# Autodesk Inventor assembly: 200-60-DIFFERENTIAL-BAR-02
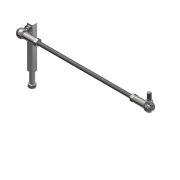
[picture p0: Inventor's stored thumbnail of the model, 180x180]
Saved by Autodesk Inventor 2018.2 (Build 222227000, 227)
## iProperties
Created: 2017-12-18
Part Number: 200-60-DIFFERENTIAL-BAR-02
Document SubType Name: Assembly
Designer: feesmrt
Author: feesmrt
## Documents named in this file (6)
- D:\Programmierung\FRANC0R\CAD\02-Rocker-Bogie-Robot\200-ROCKER-BOGIE\200-60-DIFFERENTIAL\200-60-DIFFERENTIAL-BAR-02.iam
- D:\Programmierung\FRANC0R\CAD\02-Rocker-Bogie-Robot\200-ROCKER-BOGIE\200-60-DIFFERENTIAL\200-60-DIFFERENTIAL-BAR-01.ipt
- D:\Programmierung\FRANC0R\CAD\02-Rocker-Bogie-Robot\900-COMPONENTS\900-41-NUTS\900-41-NUTS-ISO4033-M6.ipt
- D:\Programmierung\FRANC0R\CAD\02-Rocker-Bogie-Robot\900-COMPONENTS\900-70-ANGLE-JOINTS\900-70-ANGLE-JOINTS-DIN71802-M6.ipt
- D:\Programmierung\FRANC0R\CAD\02-Rocker-Bogie-Robot\900-COMPONENTS\900-80-WASHERS\900-80-WASHERS-ISO8738-6.ipt
- D:\Programmierung\FRANC0R\CAD\02-Rocker-Bogie-Robot\200-ROCKER-BOGIE\200-60-DIFFERENTIAL\200-60-DIFFERENTIAL-BAR-02.ipt
## Components (9 placed, 5 different names)
1. 200-60-DIFFERENTIAL-BAR-01:1 — Passend:1, Passend:2, Passend:3, Winkel:1, Passend:8, Winkel:2
2. 900-41-NUTS-ISO4033-M6:1 — Passend:1, Passend:2
3. 900-70-ANGLE-JOINTS-DIN71802-M6:1 — Passend:3, Passend:4, Passend:5, Winkel:1, Passend:9, Passend:10, Passend:12
4. 900-80-WASHERS-ISO8738-6:1 — Passend:7, Passend:8
5. 900-80-WASHERS-ISO8738-6:2 — Passend:4, Passend:5, Passend:7
6. 200-60-DIFFERENTIAL-BAR-02:1 — Passend:9, Passend:10, Passend:11, Passend:13, Passend:14, Passend:15
7. 900-41-NUTS-ISO4033-M6:2 — Passend:11, Passend:12
8. 900-41-NUTS-ISO4033-M6:3 — Passend:15, Passend:16
9. 900-70-ANGLE-JOINTS-DIN71802-M6:2 — Passend:13, Passend:14, Winkel:2, Passend:16
## Relationships (17: Mate 15, Angle 2)
- Passend:1 [Mate]: 200-60-DIFFERENTIAL-BAR-01:1 ↔ 900-41-NUTS-ISO4033-M6:1
- Passend:2 [Mate] (20 mm): 200-60-DIFFERENTIAL-BAR-01:1 ↔ 900-41-NUTS-ISO4033-M6:1
- Passend:3 [Mate]: 200-60-DIFFERENTIAL-BAR-01:1 ↔ 900-70-ANGLE-JOINTS-DIN71802-M6:1
- Passend:4 [Mate]: 900-70-ANGLE-JOINTS-DIN71802-M6:1 ↔ 900-80-WASHERS-ISO8738-6:2
- Passend:5 [Mate]: 900-70-ANGLE-JOINTS-DIN71802-M6:1 ↔ 900-80-WASHERS-ISO8738-6:2
- Passend:7 [Mate]: 900-80-WASHERS-ISO8738-6:1 ↔ 900-80-WASHERS-ISO8738-6:2
- Winkel:1 [Angle] (180 deg): 200-60-DIFFERENTIAL-BAR-01:1 ↔ 900-70-ANGLE-JOINTS-DIN71802-M6:1
- Passend:8 [Mate]: 200-60-DIFFERENTIAL-BAR-01:1 ↔ 900-80-WASHERS-ISO8738-6:1
- Passend:9 [Mate]: 900-70-ANGLE-JOINTS-DIN71802-M6:1 ↔ 200-60-DIFFERENTIAL-BAR-02:1
- Passend:10 [Mate] (-10 mm): 900-70-ANGLE-JOINTS-DIN71802-M6:1 ↔ 200-60-DIFFERENTIAL-BAR-02:1
- Passend:11 [Mate]: 200-60-DIFFERENTIAL-BAR-02:1 ↔ 900-41-NUTS-ISO4033-M6:2
- Passend:12 [Mate]: 900-70-ANGLE-JOINTS-DIN71802-M6:1 ↔ 900-41-NUTS-ISO4033-M6:2
- Passend:13 [Mate]: 200-60-DIFFERENTIAL-BAR-02:1 ↔ 900-70-ANGLE-JOINTS-DIN71802-M6:2
- Passend:14 [Mate] (-10 mm): 200-60-DIFFERENTIAL-BAR-02:1 ↔ 900-70-ANGLE-JOINTS-DIN71802-M6:2
- Winkel:2 [Angle] (0 deg): 200-60-DIFFERENTIAL-BAR-01:1 ↔ 900-70-ANGLE-JOINTS-DIN71802-M6:2
- Passend:15 [Mate]: 200-60-DIFFERENTIAL-BAR-02:1 ↔ 900-41-NUTS-ISO4033-M6:3
- Passend:16 [Mate]: 900-41-NUTS-ISO4033-M6:3 ↔ 900-70-ANGLE-JOINTS-DIN71802-M6:2
